# Autodesk Inventor assembly: Chassis-ver4-1111-2019
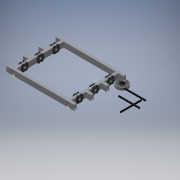
[picture p0: Inventor's stored thumbnail of the model, 180x180]
Saved by Autodesk Inventor 2018 (Build 220112000, 112)
## iProperties
Created: 2019-10-10
Part Number: Chassis-ver4-1111-2019
Document SubType Name: Assembly
Designer: JMHal
Author: JMHal
## Documents named in this file (8)
- E:\GrabCad\2019 - 2020 Off Season\TestChassis\Assembly\Chassis-ver4-1111-2019.iam
- E:\GrabCad\2019 - 2020 Off Season\TestChassis\Parts\2x1 20in Alluminum with Cal Drop.ver1-1111-2019.ipt
- E:\GrabCad\2019 - 2020 Off Season\TestChassis\Parts\2x1 20in Alluminum.ver1-1111-2019.ipt
- E:\GrabCad\2019 - 2020 Off Season\TestChassis\Parts\2x1 2in Alluminum Block.ver1-1111-2019.ipt
- E:\GrabCad\Resources\VEXpro Resources\Bearings\0.5inHexFlangedBearing(1.125inx0.313in)-1111-2016.ipt
- E:\GrabCad\Resources\VEXpro Resources\Versa Motion\VersaBlockKit-1111-2016.ipt
- E:\GrabCad\Resources\VEXpro Resources\Wheels\4 inch\4x1inTractionWheel(Tire)-1111-2016.iam
- E:\GrabCad\Resources\VEXpro Resources\Shafts\0.5inThunderHexShaft(8)-1111-2016.ipt
## Components (40 placed, 7 different names)
1. 2x1 20in Alluminum with Cal Drop.ver1-1111-2019:1 — Mate:1, Mate:2, Mate:19, Mate:20, Mate:21, Mate:28, Mate:29, Mate:30, Mate:31, Mate:32, Mate:33, Mate:34, Mate:41, Mate:42, Rotational:1, Angle:1, Insert:6, Insert:7, Mate:51, Insert:8, Angle:2, Mate:53, Angle:9, Insert:17, Angle:10, Insert:19, Angle:11, Insert:21, Angle:12
2. 2x1 20in Alluminum.ver1-1111-2019:1 — Mate:1, Mate:2, Mate:3, Mate:5, Mate:6
3. 2x1 20in Alluminum with Cal Drop.ver1-1111-2019:2 — Mate:3, Mate:5, Mate:6, Mate:7, Mate:8, Mate:9, Mate:22, Mate:23, Mate:24, Mate:25, Mate:26, Mate:27, Mate:35, Mate:36, Mate:37, Mate:38, Mate:39, Mate:40, Insert:3, Insert:4, Insert:5, Angle:6, Angle:7, Angle:8, Insert:23, Angle:13, Insert:25, Angle:14, Insert:27, Angle:15
4. 2x1 20in Alluminum.ver1-1111-2019:2 — Mate:7, Mate:8, Mate:9
5. 2x1 2in Alluminum Block.ver1-1111-2019:1 — Mate:22, Mate:23, Mate:24
6. 2x1 2in Alluminum Block.ver1-1111-2019:2 — Mate:19, Mate:20, Mate:21
7. 2x1 2in Alluminum Block.ver1-1111-2019:3 — Mate:25, Mate:26, Mate:27
8. 2x1 2in Alluminum Block.ver1-1111-2019:4 — Mate:28, Mate:29, Mate:30
9. 2x1 2in Alluminum Block.ver1-1111-2019:5 — Mate:31, Mate:32, Mate:41
10. 2x1 2in Alluminum Block.ver1-1111-2019:6 — Mate:33, Mate:34, Mate:42
11. 2x1 2in Alluminum Block.ver1-1111-2019:7 — Mate:35, Mate:36, Mate:40
12. 2x1 2in Alluminum Block.ver1-1111-2019:8 — Mate:37, Mate:38, Mate:39
13. VersaBlockKit-1111-2016:1 — Mate:44, Mate:45, Angle:6
14. 0.5inHexFlangedBearing(1.125inx0.313in)-1111-2016:5 — Insert:3, Mate:44, Mate:45
15. 0.5inHexFlangedBearing(1.125inx0.313in)-1111-2016:6 — Insert:4, Mate:46, Mate:47
16. VersaBlockKit-1111-2016:2 — Mate:46, Mate:47, Angle:8
17. 0.5inHexFlangedBearing(1.125inx0.313in)-1111-2016:7 — Insert:5, Mate:48, Mate:49
18. VersaBlockKit-1111-2016:3 — Mate:48, Mate:49, Angle:7
19. VersaBlockKit-1111-2016:4 — Rotational:1, Angle:1
20. 0.5inHexFlangedBearing(1.125inx0.313in)-1111-2016:8 — Insert:6
21. 0.5inHexFlangedBearing(1.125inx0.313in)-1111-2016:9 — Insert:7, Mate:50
22. VersaBlockKit-1111-2016:5 — Mate:50, Mate:51, Angle:2
23. 0.5inHexFlangedBearing(1.125inx0.313in)-1111-2016:10 — Insert:8, Mate:52
24. VersaBlockKit-1111-2016:6 — Mate:52, Mate:53, Angle:9
25. 4x1inTractionWheel(Tire)-1111-2016:1 [sub-assembly]
26. 0.5inThunderHexShaft(8)-1111-2016:1
27. 0.5inThunderHexShaft(8)-1111-2016:2
28. 0.5inThunderHexShaft(8)-1111-2016:3
29. 0.5inHexFlangedBearing(1.125inx0.313in)-1111-2016:16 — Insert:16, Insert:17
30. VersaBlockKit-1111-2016:8 — Insert:16, Angle:10
31. 0.5inHexFlangedBearing(1.125inx0.313in)-1111-2016:17 — Insert:19
32. VersaBlockKit-1111-2016:9 — Angle:11
33. 0.5inHexFlangedBearing(1.125inx0.313in)-1111-2016:18
34. VersaBlockKit-1111-2016:10 — Insert:21, Angle:12
35. 0.5inHexFlangedBearing(1.125inx0.313in)-1111-2016:19
36. VersaBlockKit-1111-2016:11 — Insert:23, Angle:13
37. 0.5inHexFlangedBearing(1.125inx0.313in)-1111-2016:20
38. VersaBlockKit-1111-2016:12 — Insert:25, Angle:14
39. 0.5inHexFlangedBearing(1.125inx0.313in)-1111-2016:21
40. VersaBlockKit-1111-2016:13 — Insert:27, Angle:15
## Relationships (79: Mate 48, Insert 18, Angle 12, RevoluteJoint 1)
- Mate:1: 2x1 20in Alluminum with Cal Drop.ver1-1111-2019:1 ↔ 2x1 20in Alluminum.ver1-1111-2019:1
- Mate:2: 2x1 20in Alluminum with Cal Drop.ver1-1111-2019:1 ↔ 2x1 20in Alluminum.ver1-1111-2019:1
- Mate:3: 2x1 20in Alluminum.ver1-1111-2019:1 ↔ 2x1 20in Alluminum with Cal Drop.ver1-1111-2019:2
- Mate:5: 2x1 20in Alluminum.ver1-1111-2019:1 ↔ 2x1 20in Alluminum with Cal Drop.ver1-1111-2019:2
- Mate:6: 2x1 20in Alluminum.ver1-1111-2019:1 ↔ 2x1 20in Alluminum with Cal Drop.ver1-1111-2019:2
- Mate:7: 2x1 20in Alluminum with Cal Drop.ver1-1111-2019:2 ↔ 2x1 20in Alluminum.ver1-1111-2019:2
- Mate:8: 2x1 20in Alluminum with Cal Drop.ver1-1111-2019:2 ↔ 2x1 20in Alluminum.ver1-1111-2019:2
- Mate:9: 2x1 20in Alluminum with Cal Drop.ver1-1111-2019:2 ↔ 2x1 20in Alluminum.ver1-1111-2019:2
- Mate:19: 2x1 20in Alluminum with Cal Drop.ver1-1111-2019:1 ↔ 2x1 2in Alluminum Block.ver1-1111-2019:2
- Mate:20: 2x1 20in Alluminum with Cal Drop.ver1-1111-2019:1 ↔ 2x1 2in Alluminum Block.ver1-1111-2019:2
- Mate:21: 2x1 20in Alluminum with Cal Drop.ver1-1111-2019:1 ↔ 2x1 2in Alluminum Block.ver1-1111-2019:2
- Mate:22: 2x1 20in Alluminum with Cal Drop.ver1-1111-2019:2 ↔ 2x1 2in Alluminum Block.ver1-1111-2019:1
- Mate:23: 2x1 20in Alluminum with Cal Drop.ver1-1111-2019:2 ↔ 2x1 2in Alluminum Block.ver1-1111-2019:1
- Mate:24: 2x1 20in Alluminum with Cal Drop.ver1-1111-2019:2 ↔ 2x1 2in Alluminum Block.ver1-1111-2019:1
- Mate:25: 2x1 20in Alluminum with Cal Drop.ver1-1111-2019:2 ↔ 2x1 2in Alluminum Block.ver1-1111-2019:3
- Mate:26: 2x1 20in Alluminum with Cal Drop.ver1-1111-2019:2 ↔ 2x1 2in Alluminum Block.ver1-1111-2019:3
- Mate:27: 2x1 20in Alluminum with Cal Drop.ver1-1111-2019:2 ↔ 2x1 2in Alluminum Block.ver1-1111-2019:3
- Mate:28: 2x1 20in Alluminum with Cal Drop.ver1-1111-2019:1 ↔ 2x1 2in Alluminum Block.ver1-1111-2019:4
- Mate:29: 2x1 20in Alluminum with Cal Drop.ver1-1111-2019:1 ↔ 2x1 2in Alluminum Block.ver1-1111-2019:4
- Mate:30: 2x1 20in Alluminum with Cal Drop.ver1-1111-2019:1 ↔ 2x1 2in Alluminum Block.ver1-1111-2019:4
- Mate:31: 2x1 20in Alluminum with Cal Drop.ver1-1111-2019:1 ↔ 2x1 2in Alluminum Block.ver1-1111-2019:5
- Mate:32: 2x1 20in Alluminum with Cal Drop.ver1-1111-2019:1 ↔ 2x1 2in Alluminum Block.ver1-1111-2019:5
- Mate:33: 2x1 20in Alluminum with Cal Drop.ver1-1111-2019:1 ↔ 2x1 2in Alluminum Block.ver1-1111-2019:6
- Mate:34: 2x1 20in Alluminum with Cal Drop.ver1-1111-2019:1 ↔ 2x1 2in Alluminum Block.ver1-1111-2019:6
- Mate:35: 2x1 20in Alluminum with Cal Drop.ver1-1111-2019:2 ↔ 2x1 2in Alluminum Block.ver1-1111-2019:7
- Mate:36: 2x1 20in Alluminum with Cal Drop.ver1-1111-2019:2 ↔ 2x1 2in Alluminum Block.ver1-1111-2019:7
- Mate:37: 2x1 20in Alluminum with Cal Drop.ver1-1111-2019:2 ↔ 2x1 2in Alluminum Block.ver1-1111-2019:8
- Mate:38: 2x1 20in Alluminum with Cal Drop.ver1-1111-2019:2 ↔ 2x1 2in Alluminum Block.ver1-1111-2019:8
- Mate:39 (63.5 mm): 2x1 20in Alluminum with Cal Drop.ver1-1111-2019:2 ↔ 2x1 2in Alluminum Block.ver1-1111-2019:8
- Mate:40 (63.5 mm): 2x1 20in Alluminum with Cal Drop.ver1-1111-2019:2 ↔ 2x1 2in Alluminum Block.ver1-1111-2019:7
- Mate:41 (63.5 mm): 2x1 20in Alluminum with Cal Drop.ver1-1111-2019:1 ↔ 2x1 2in Alluminum Block.ver1-1111-2019:5
- Mate:42 (63.5 mm): 2x1 20in Alluminum with Cal Drop.ver1-1111-2019:1 ↔ 2x1 2in Alluminum Block.ver1-1111-2019:6
- Insert:3: 2x1 20in Alluminum with Cal Drop.ver1-1111-2019:2 ↔ 0.5inHexFlangedBearing(1.125inx0.313in)-1111-2016:5
- Mate:44: VersaBlockKit-1111-2016:1 ↔ 0.5inHexFlangedBearing(1.125inx0.313in)-1111-2016:5
- Mate:45: VersaBlockKit-1111-2016:1 ↔ 0.5inHexFlangedBearing(1.125inx0.313in)-1111-2016:5
- Insert:4: 2x1 20in Alluminum with Cal Drop.ver1-1111-2019:2 ↔ 0.5inHexFlangedBearing(1.125inx0.313in)-1111-2016:6
- Mate:46: 0.5inHexFlangedBearing(1.125inx0.313in)-1111-2016:6 ↔ VersaBlockKit-1111-2016:2
- Mate:47: 0.5inHexFlangedBearing(1.125inx0.313in)-1111-2016:6 ↔ VersaBlockKit-1111-2016:2
- Insert:5: 2x1 20in Alluminum with Cal Drop.ver1-1111-2019:2 ↔ 0.5inHexFlangedBearing(1.125inx0.313in)-1111-2016:7
- Mate:48: 0.5inHexFlangedBearing(1.125inx0.313in)-1111-2016:7 ↔ VersaBlockKit-1111-2016:3
- Mate:49: 0.5inHexFlangedBearing(1.125inx0.313in)-1111-2016:7 ↔ VersaBlockKit-1111-2016:3
- Rotational:1 [RevoluteJoint]: 2x1 20in Alluminum with Cal Drop.ver1-1111-2019:1 ↔ VersaBlockKit-1111-2016:4
- Angle:1 (0 deg): 2x1 20in Alluminum with Cal Drop.ver1-1111-2019:1 ↔ VersaBlockKit-1111-2016:4
- Insert:6: 2x1 20in Alluminum with Cal Drop.ver1-1111-2019:1 ↔ 0.5inHexFlangedBearing(1.125inx0.313in)-1111-2016:8
- Insert:7: 2x1 20in Alluminum with Cal Drop.ver1-1111-2019:1 ↔ 0.5inHexFlangedBearing(1.125inx0.313in)-1111-2016:9
- Mate:50: 0.5inHexFlangedBearing(1.125inx0.313in)-1111-2016:9 ↔ VersaBlockKit-1111-2016:5
- Mate:51: 2x1 20in Alluminum with Cal Drop.ver1-1111-2019:1 ↔ VersaBlockKit-1111-2016:5
- Insert:8: 2x1 20in Alluminum with Cal Drop.ver1-1111-2019:1 ↔ 0.5inHexFlangedBearing(1.125inx0.313in)-1111-2016:10
- Angle:2 (0 deg): 2x1 20in Alluminum with Cal Drop.ver1-1111-2019:1 ↔ VersaBlockKit-1111-2016:5
- Angle:6 (0 deg): 2x1 20in Alluminum with Cal Drop.ver1-1111-2019:2 ↔ VersaBlockKit-1111-2016:1
- Angle:7 (0 deg): 2x1 20in Alluminum with Cal Drop.ver1-1111-2019:2 ↔ VersaBlockKit-1111-2016:3
- Angle:8 (0 deg): 2x1 20in Alluminum with Cal Drop.ver1-1111-2019:2 ↔ VersaBlockKit-1111-2016:2
- Mate:52: 0.5inHexFlangedBearing(1.125inx0.313in)-1111-2016:10 ↔ VersaBlockKit-1111-2016:6
- Mate:53: 2x1 20in Alluminum with Cal Drop.ver1-1111-2019:1 ↔ VersaBlockKit-1111-2016:6
- Angle:9 (0 deg): 2x1 20in Alluminum with Cal Drop.ver1-1111-2019:1 ↔ VersaBlockKit-1111-2016:6
- [Mate]: 0.5inHexFlangedBearing(1.125inx0.313in)-1111-2016:16 ↔ VersaBlockKit-1111-2016:8
- Insert:16: 0.5inHexFlangedBearing(1.125inx0.313in)-1111-2016:16 ↔ VersaBlockKit-1111-2016:8
- Insert:17: 2x1 20in Alluminum with Cal Drop.ver1-1111-2019:1 ↔ 0.5inHexFlangedBearing(1.125inx0.313in)-1111-2016:16
- Angle:10 (0 deg): 2x1 20in Alluminum with Cal Drop.ver1-1111-2019:1 ↔ VersaBlockKit-1111-2016:8
- [Mate]: 0.5inHexFlangedBearing(1.125inx0.313in)-1111-2016:17 ↔ VersaBlockKit-1111-2016:9
- [Insert]: 0.5inHexFlangedBearing(1.125inx0.313in)-1111-2016:17 ↔ VersaBlockKit-1111-2016:9
- Insert:19: 2x1 20in Alluminum with Cal Drop.ver1-1111-2019:1 ↔ 0.5inHexFlangedBearing(1.125inx0.313in)-1111-2016:17
- Angle:11 (0 deg): 2x1 20in Alluminum with Cal Drop.ver1-1111-2019:1 ↔ VersaBlockKit-1111-2016:9
- [Mate]: 0.5inHexFlangedBearing(1.125inx0.313in)-1111-2016:18 ↔ VersaBlockKit-1111-2016:10
- [Insert]: 0.5inHexFlangedBearing(1.125inx0.313in)-1111-2016:18 ↔ VersaBlockKit-1111-2016:10
- Insert:21: 2x1 20in Alluminum with Cal Drop.ver1-1111-2019:1 ↔ VersaBlockKit-1111-2016:10
- Angle:12 (0 deg): 2x1 20in Alluminum with Cal Drop.ver1-1111-2019:1 ↔ VersaBlockKit-1111-2016:10
- [Mate]: 0.5inHexFlangedBearing(1.125inx0.313in)-1111-2016:19 ↔ VersaBlockKit-1111-2016:11
- [Insert]: 0.5inHexFlangedBearing(1.125inx0.313in)-1111-2016:19 ↔ VersaBlockKit-1111-2016:11
- Insert:23: 2x1 20in Alluminum with Cal Drop.ver1-1111-2019:2 ↔ VersaBlockKit-1111-2016:11
- Angle:13 (0 deg): 2x1 20in Alluminum with Cal Drop.ver1-1111-2019:2 ↔ VersaBlockKit-1111-2016:11
- [Mate]: 0.5inHexFlangedBearing(1.125inx0.313in)-1111-2016:20 ↔ VersaBlockKit-1111-2016:12
- [Insert]: 0.5inHexFlangedBearing(1.125inx0.313in)-1111-2016:20 ↔ VersaBlockKit-1111-2016:12
- Insert:25: 2x1 20in Alluminum with Cal Drop.ver1-1111-2019:2 ↔ VersaBlockKit-1111-2016:12
- Angle:14 (0 deg): 2x1 20in Alluminum with Cal Drop.ver1-1111-2019:2 ↔ VersaBlockKit-1111-2016:12
- [Mate]: 0.5inHexFlangedBearing(1.125inx0.313in)-1111-2016:21 ↔ VersaBlockKit-1111-2016:13
- [Insert]: 0.5inHexFlangedBearing(1.125inx0.313in)-1111-2016:21 ↔ VersaBlockKit-1111-2016:13
- Insert:27: 2x1 20in Alluminum with Cal Drop.ver1-1111-2019:2 ↔ VersaBlockKit-1111-2016:13
- Angle:15 (0 deg): 2x1 20in Alluminum with Cal Drop.ver1-1111-2019:2 ↔ VersaBlockKit-1111-2016:13
## Named parameters: d89_d76 = 0 mm, d93_d89_d76 = 0 mm, d94_d90 = 0 mm, d99_d89_d76 = 0 mm, d100_d90 = 0 mm, d103_d89_d76 = 0 mm, d104_d90 = 0 mm, d107_d89_d76 = 0 mm, d108_d90 = 0 mm, d111_d89_d76 = 0 mm, d112_d90 = 0 mm
